# Autodesk Inventor assembly: frame
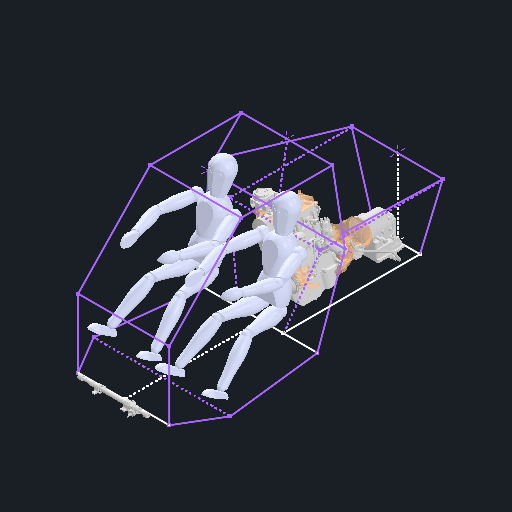
[picture p0: Inventor's stored thumbnail of the model, 512x512]
Saved by Autodesk Inventor 2025.3 (Build 293356000, 356)
## iProperties
Created: 2026-09-23
Part Number: frame
Document SubType Name: Assembly
Designer: VianaCC
Author: VianaCC
## Documents named in this file (5)
- C:\Users\vianacc\Documents\GitHub\utv_startup\products\utv\chassis\cad\draft\frame.iam
- C:\Users\vianacc\Documents\GitHub\utv_startup\products\utv\powertrain\cad\reference\motor-volkswagen-ap-1800-cc-de-1\Paulo R Conjunto MOTOR VW AP 1800 - 1998\Paulo R Conjunto MOTOR VW AP 1800 - 1998\Paulo R Con.iam
- C:\Users\vianacc\Documents\GitHub\utv_startup\products\utv\chassis\cad\draft\frame_skel.ipt
- C:\Users\vianacc\Documents\GitHub\utv_startup\products\utv\ergonomics\cad\reference\maniac.iam
- C:\Users\vianacc\Documents\GitHub\utv_startup\products\utv\steering\cad\reference\Ford escort mk 1 & 2 steering rack\Ford escort mk 1 & 2 steering rack\Ford escort mk 1 & 2 steering rack.iam
## Components (5 placed, 4 different names)
1. Paulo R Con:1 [sub-assembly]
2. frame_skel:1 — Mate:5
3. maniac:1 [sub-assembly] — Mate:6, Mate:7, Mate:8, Angle:1
4. maniac:2 [sub-assembly] — Mate:9, Mate:10, Mate:11
5. Ford escort mk 1 & 2 steering rack:1 [sub-assembly] — Flush:13
## Relationships (9: Mate 7, Angle 1, Flush 1)
- Mate:5: frame_skel:1
- Mate:6 (400 mm): maniac:1
- Mate:7 (300 mm): maniac:1
- Mate:8 (1400 mm): maniac:1
- Angle:1 (180 deg): maniac:1
- Mate:9 (400 mm): maniac:2
- Mate:10 (1400 mm): maniac:2
- Mate:11 (-300 mm): maniac:2
- Flush:13: Ford escort mk 1 & 2 steering rack:1
